# Autodesk Inventor assembly: MPG Assy
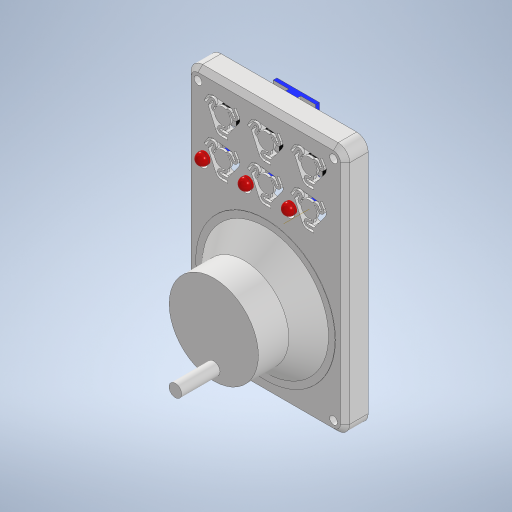
[picture p0: Inventor's stored thumbnail of the model, 512x512]
Saved by Autodesk Inventor 2023.1 (Build 271208000, 208)
## iProperties
Created: 2022-10-09
Part Number: MPG Assy
Document SubType Name: Assembly
Designer: Nick
Author: Nick
## Documents named in this file (8)
- Y:\Projects\CNC_MPG\MPG Assy.iam
- Y:\Projects\CNC_MPG\Arduino Pro Micro.ipt
- Y:\Projects\CNC_MPG\Button.ipt
- Y:\Projects\CNC_MPG\Case Back.ipt
- Y:\Projects\CNC_MPG\Case Front.ipt
- Y:\Projects\CNC_MPG\MPG.ipt
- Y:\Projects\CNC_MPG\LED.ipt
- Y:\Projects\CNC_MPG\Button Support.ipt
## Components (15 placed, 7 different names)
1. Arduino Pro Micro:1 — Mate:3, Mate:4, Mate:5
2. Case Front:1 — Insert:1, Insert:2, Insert:3, Insert:4, Insert:5, Insert:6, Insert:7, Insert:8, Insert:9, Insert:10, Mate:1, Flush:1, Flush:2
3. MPG:1 — Insert:1
4. Button:4 — Insert:2
5. Button:5 — Insert:3
6. Button:6 — Insert:5, Mate:6, Flush:3, Mate:7
7. Button:7 — Insert:6
8. Button:8 — Insert:4
9. Button:9 — Insert:7, Mate:8, Flush:4, Mate:9
10. LED:1 — Insert:8
11. LED:2 — Insert:9
12. LED:3 — Insert:10
13. Case Back:1 — Mate:1, Flush:1, Flush:2, Mate:3, Mate:4, Mate:5
14. Button Support:1 — Mate:6, Flush:3, Mate:7
15. Button Support:2 — Mate:8, Flush:4, Mate:9
## Relationships (22: Insert 10, Mate 8, Flush 4)
- Insert:1: Case Front:1 ↔ MPG:1
- Insert:2: Case Front:1 ↔ Button:4
- Insert:3: Case Front:1 ↔ Button:5
- Insert:4: Case Front:1 ↔ Button:8
- Insert:5: Case Front:1 ↔ Button:6
- Insert:6: Case Front:1 ↔ Button:7
- Insert:7: Case Front:1 ↔ Button:9
- Insert:8: Case Front:1 ↔ LED:1
- Insert:9: Case Front:1 ↔ LED:2
- Insert:10: Case Front:1 ↔ LED:3
- Mate:1: Case Front:1 ↔ Case Back:1
- Flush:1: Case Front:1 ↔ Case Back:1
- Flush:2: Case Front:1 ↔ Case Back:1
- Mate:3: Arduino Pro Micro:1 ↔ Case Back:1
- Mate:4: Arduino Pro Micro:1 ↔ Case Back:1
- Mate:5: Arduino Pro Micro:1 ↔ Case Back:1
- Mate:6: Button:6 ↔ Button Support:1
- Flush:3: Button:6 ↔ Button Support:1
- Mate:7: Button:6 ↔ Button Support:1
- Mate:8: Button:9 ↔ Button Support:2
- Flush:4: Button:9 ↔ Button Support:2
- Mate:9: Button:9 ↔ Button Support:2
